# Autodesk Inventor assembly: s-assy-sorter_motor
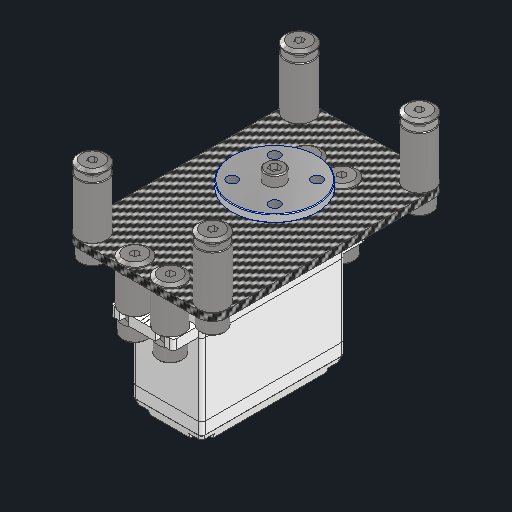
[picture p0: Inventor's stored thumbnail of the model, 512x512]
Saved by Autodesk Inventor 2022 (Build 260153000, 153)
## iProperties
Created: 2021-08-27
Part Number: s-assy-sorter_motor
Document SubType Name: Assembly
Designer: Yuta Kage
Author: Yuta Kage
## Documents named in this file (8)
- C:\Users\yuta0\Desktop\catchrobo_shooter\s-assy-sorter_motor.iam
- C:\Users\yuta0\Desktop\catchrobo_shooter\MG_996R.iam
- C:\Users\yuta0\Desktop\catchrobo_shooter\ARF-410E.ipt
- C:\Users\yuta0\Desktop\catchrobo_shooter\CB4-6.ipt
- C:\Users\yuta0\Desktop\catchrobo_shooter\CBSTSR4-6.ipt
- C:\Users\yuta0\Desktop\catchrobo_shooter\CB3-5.ipt
- C:\Users\yuta0\Desktop\catchrobo_shooter\ARF-415.ipt
- C:\Users\yuta0\Desktop\catchrobo_shooter\shooter_carbon_plate3.ipt
## Components (27 placed, 7 different names)
1. shooter_carbon_plate3:1 — メイト:58, メイト:60, メイト:61, メイト:62, メイト:63, メイト:66, メイト:69, メイト:71
2. MG_996R:1 [sub-assembly] — メイト:22, メイト:56, メイト:57, メイト:61, メイト:64, メイト:65
3. CB3-5:1 — メイト:64, メイト:65
4. ARF-410E:2 — メイト:22, メイト:58, メイト:60
5. CB4-6:9 — メイト:56, メイト:57
6. CBSTSR4-6:1 — メイト:62, メイト:63
7. ARF-410E:3
8. CB4-6:10
9. CBSTSR4-6:2
10. ARF-410E:4
11. CB4-6:11
12. CBSTSR4-6:3
13. ARF-410E:5
14. CB4-6:12
15. CBSTSR4-6:4
16. ARF-415:1 — メイト:67, メイト:68, メイト:70, メイト:71, メイト:72
17. CBSTSR4-6:5 — メイト:68, メイト:72
18. CB4-6:13 — メイト:66, メイト:67, メイト:69, メイト:70
19. ARF-415:2
20. CBSTSR4-6:6
21. CB4-6:14
22. ARF-415:3
23. CBSTSR4-6:7
24. CB4-6:15
25. ARF-415:4
26. CBSTSR4-6:8
27. CB4-6:16
## Component patterns: (4 elements, first: ARF-410E:2 + CB4-6:9 + CBSTSR4-6:1), (4 elements, first: ARF-415:1 + CBSTSR4-6:5 + CB4-6:13)
## Relationships (17: Mate 17)
- メイト:22 [Mate]: MG_996R:1 ↔ ARF-410E:2
- メイト:56 [Mate]: MG_996R:1 ↔ CB4-6:9
- メイト:57 [Mate]: MG_996R:1 ↔ CB4-6:9
- メイト:58 [Mate]: shooter_carbon_plate3:1 ↔ ARF-410E:2
- メイト:60 [Mate]: shooter_carbon_plate3:1 ↔ ARF-410E:2
- メイト:61 [Mate]: shooter_carbon_plate3:1 ↔ MG_996R:1
- メイト:62 [Mate]: shooter_carbon_plate3:1 ↔ CBSTSR4-6:1
- メイト:63 [Mate]: shooter_carbon_plate3:1 ↔ CBSTSR4-6:1
- メイト:64 [Mate]: MG_996R:1 ↔ CB3-5:1
- メイト:65 [Mate]: MG_996R:1 ↔ CB3-5:1
- メイト:66 [Mate]: shooter_carbon_plate3:1 ↔ CB4-6:13
- メイト:67 [Mate]: ARF-415:1 ↔ CB4-6:13
- メイト:68 [Mate]: ARF-415:1 ↔ CBSTSR4-6:5
- メイト:69 [Mate]: shooter_carbon_plate3:1 ↔ CB4-6:13
- メイト:70 [Mate]: ARF-415:1 ↔ CB4-6:13
- メイト:71 [Mate]: shooter_carbon_plate3:1 ↔ ARF-415:1
- メイト:72 [Mate] (2 mm): ARF-415:1 ↔ CBSTSR4-6:5
